# Autodesk Inventor assembly: OmniWheel
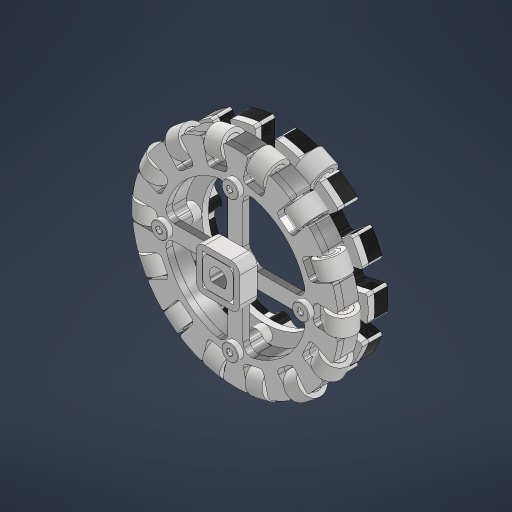
[picture p0: Inventor's stored thumbnail of the model, 512x512]
Saved by Autodesk Inventor 2024.2 (Build 282272000, 272)
## iProperties
Created: 2023-12-20
Part Number: OmniWheel
Document SubType Name: Assembly
Designer: Hanaoka
Author: Hanaoka
## Documents named in this file (8)
- G:\共有ドライブ\reRo\05_個人\hanaoka\inventor\DriveUnit\OmniWheel.iam
- G:\共有ドライブ\reRo\05_個人\hanaoka\inventor\DriveUnit\OmniFrame_B.ipt
- G:\共有ドライブ\reRo\05_個人\hanaoka\inventor\DriveUnit\SideWheel.iam
- G:\共有ドライブ\reRo\05_個人\hanaoka\inventor\DriveUnit\OmniFrame_A.ipt
- G:\共有ドライブ\reRo\05_個人\hanaoka\inventor\CAMpath\Tap_zigu.ipt
- G:\共有ドライブ\reRo\05_個人\hanaoka\inventor\DriveUnit\OmniFrame_D.ipt
- G:\共有ドライブ\reRo\05_個人\hanaoka\inventor\DriveUnit\OmniFrame_C.ipt
- G:\共有ドライブ\reRo\05_個人\hanaoka\inventor\Screw\M2xL6\M2x6.ipt
## Components (24 placed, 7 different names)
1. OmniFrame_B:1 — メイト:2, メイト:3, メイト:4, メイト:5, 正接:2, 正接:3, 挿入:4, 挿入:12
2. OmniFrame_A:1 — フラッシュ:1, 正接:1, メイト:1, メイト:2, メイト:3, メイト:4, フラッシュ:2, 挿入:8, 挿入:9, 挿入:10, 挿入:11
3. Tap_zigu:1 — フラッシュ:2
4. OmniFrame_D:1 — 挿入:13, 挿入:14, 正接:4, メイト:6
5. OmniFrame_C:1 — 挿入:4, 挿入:12, 挿入:13, 挿入:14, 正接:5
6. M2x6:1 — 挿入:11
7. M2x6:2 — 挿入:10
8. M2x6:3 — 挿入:9
9. M2x6:4 — 挿入:8
10. SideWheel:15 [sub-assembly] — 正接:4, メイト:6, 正接:5
11. SideWheel:1 [sub-assembly] — メイト:5, 正接:2, 正接:3
12. SideWheel:2 [sub-assembly]
13. SideWheel:3 [sub-assembly]
14. SideWheel:4 [sub-assembly]
15. SideWheel:5 [sub-assembly]
16. SideWheel:6 [sub-assembly]
17. SideWheel:7 [sub-assembly]
18. SideWheel:8 [sub-assembly]
19. SideWheel:9 [sub-assembly]
20. SideWheel:10 [sub-assembly]
21. SideWheel:11 [sub-assembly]
22. SideWheel:12 [sub-assembly]
23. SideWheel:13 [sub-assembly]
24. SideWheel:14 [sub-assembly]
## Component patterns: (14 elements, first: SideWheel:1)
## Relationships (21: Insert 8, Mate 6, Tangent 5, Flush 2)
- フラッシュ:1 [Flush]: OmniFrame_A:1
- 正接:1 [Tangent]: OmniFrame_A:1
- メイト:1 [Mate] (6 mm): OmniFrame_A:1
- メイト:2 [Mate]: OmniFrame_B:1 ↔ OmniFrame_A:1
- メイト:3 [Mate]: OmniFrame_B:1 ↔ OmniFrame_A:1
- メイト:4 [Mate]: OmniFrame_B:1 ↔ OmniFrame_A:1
- メイト:5 [Mate] (0.25 mm): OmniFrame_B:1 ↔ SideWheel:1
- 正接:2 [Tangent] (0.025 mm): OmniFrame_B:1 ↔ SideWheel:1
- 正接:3 [Tangent] (0.025 mm): OmniFrame_B:1 ↔ SideWheel:1
- フラッシュ:2 [Flush]: OmniFrame_A:1 ↔ Tap_zigu:1
- 挿入:4 [Insert]: OmniFrame_B:1 ↔ OmniFrame_C:1
- 挿入:8 [Insert]: OmniFrame_A:1 ↔ M2x6:4
- 挿入:9 [Insert]: OmniFrame_A:1 ↔ M2x6:3
- 挿入:10 [Insert]: OmniFrame_A:1 ↔ M2x6:2
- 挿入:11 [Insert]: OmniFrame_A:1 ↔ M2x6:1
- 挿入:12 [Insert]: OmniFrame_B:1 ↔ OmniFrame_C:1
- 挿入:13 [Insert]: OmniFrame_D:1 ↔ OmniFrame_C:1
- 挿入:14 [Insert]: OmniFrame_D:1 ↔ OmniFrame_C:1
- 正接:4 [Tangent]: OmniFrame_D:1 ↔ SideWheel:15
- メイト:6 [Mate] (-0.5 mm): OmniFrame_D:1 ↔ SideWheel:15
- 正接:5 [Tangent]: OmniFrame_C:1 ↔ SideWheel:15
